# Autodesk Inventor assembly: POM_T5_1_hanakawa_221012
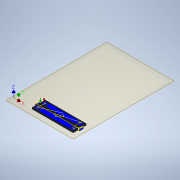
[picture p0: Inventor's stored thumbnail of the model, 180x180]
Saved by Autodesk Inventor 2022 (Build 260153000, 153)
## iProperties
Created: 2022-09-28
Part Number: POM_T5_1_hanakawa_221012
Document SubType Name: Assembly
Designer: Masato
Author: Masato
## Documents named in this file (3)
- C:\Users\hanak\Documents\SUSTAINA-OP\Cam\POM_T5\POM_T5_1_hanakawa_221012.iam
- C:\Users\hanak\Documents\SUSTAINA-OP\Cam\DisposableBoard.ipt
- C:\Users\hanak\Documents\SUSTAINA-OP\UpperBody\Cockpit\Cockpit_battery_bottom_frame.ipt
## Components (2 placed, 2 different names)
1. DisposableBoard:1 — フラッシュ:1, フラッシュ:2, フラッシュ:3, フラッシュ:4, メイト:1, フラッシュ:5, フラッシュ:6
2. Cockpit_battery_bottom_frame:1 — メイト:1, フラッシュ:5, フラッシュ:6
## Relationships (7: Flush 6, Mate 1)
- フラッシュ:1 [Flush]: DisposableBoard:1
- フラッシュ:2 [Flush]: DisposableBoard:1
- フラッシュ:3 [Flush]: DisposableBoard:1
- フラッシュ:4 [Flush]: DisposableBoard:1
- メイト:1 [Mate]: DisposableBoard:1 ↔ Cockpit_battery_bottom_frame:1
- フラッシュ:5 [Flush] (2.5 mm): DisposableBoard:1 ↔ Cockpit_battery_bottom_frame:1
- フラッシュ:6 [Flush] (2.5 mm): DisposableBoard:1 ↔ Cockpit_battery_bottom_frame:1
